# Autodesk Inventor assembly: BaseRoulante
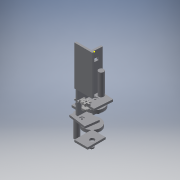
[picture p0: Inventor's stored thumbnail of the model, 180x180]
Saved by Autodesk Inventor 2017 SP1 (Build 210196100, 196)
## iProperties
Part Number: BaseRoulante
Material: Générique
Document SubType Name: Assembly
Designer: Sylvain
Author: Sylvain
## Documents named in this file (11)
- E:\1-SAUVEGARDE\Documents\Loisirs\GrosRobotOfficiel\3D\BaseRoulante.iam
- E:\1-SAUVEGARDE\Documents\Loisirs\GrosRobotOfficiel\3D\Flancs.ipt
- E:\1-SAUVEGARDE\Documents\Loisirs\GrosRobotOfficiel\3D\MoteurMaxon.ipt
- E:\1-SAUVEGARDE\Documents\Loisirs\GrosRobotOfficiel\3D\FlancExt.ipt
- E:\1-SAUVEGARDE\Documents\Loisirs\GrosRobotOfficiel\3D\Roue.ipt
- E:\1-SAUVEGARDE\Documents\Loisirs\GrosRobotOfficiel\3D\Base.ipt
- E:\1-SAUVEGARDE\Documents\Loisirs\GrosRobotOfficiel\3D\Roulement.ipt
- E:\1-SAUVEGARDE\Documents\Loisirs\GrosRobotOfficiel\3D\BaseRoulante\Design Accelerator\Engrenages cylindriques2.iam
- E:\1-SAUVEGARDE\Documents\Loisirs\GrosRobotOfficiel\3D\Toit.ipt
- E:\1-SAUVEGARDE\Documents\Loisirs\GrosRobotOfficiel\3D\BaseRoulante\Design Accelerator\Engrenages cylindriques4.iam
- E:\1-SAUVEGARDE\Documents\Loisirs\GrosRobotOfficiel\3D\BaseRoulante\Design Accelerator\Engrenages cylindriques5.iam
## Components (17 placed, 8 different names)
1. Flancs:1
2. Flancs:2 — Logement:1, Affleurement:1, Placage:1, Placage:2, Logement:3, Affleurement:2, Placage:4
3. MoteurMaxon:1 — Logement:3, Placage:3
4. MoteurMaxon:2
5. FlancExt:1
6. FlancExt:2 — Logement:2
7. Roue:1
8. Roue:2 — Cylindrique:1, Affleurement:2, Placage:5, Placage:6
9. Base:1 — Affleurement:1, Placage:1, Placage:2
10. Roulement:1 — Logement:1, Cylindrique:1
11. Roulement:2 — Logement:2
12. Roulement:3
13. Roulement:4
14. Engrenages cylindriques:1 [sub-assembly]
15. Toit:1
16. Engrenages cylindriques:2 [sub-assembly] — Placage:3, Placage:4, Placage:5, Placage:6
17. Engrenages cylindriques:3 [sub-assembly]
## Relationships (12: Mate 6, Insert 3, Flush 2, CylindricalJoint 1)
- Logement:1 [Insert]: Flancs:2 ↔ Roulement:1
- Logement:2 [Insert]: FlancExt:2 ↔ Roulement:2
- Affleurement:1 [Flush]: Flancs:2 ↔ Base:1
- Placage:1 [Mate]: Flancs:2 ↔ Base:1
- Placage:2 [Mate]: Flancs:2 ↔ Base:1
- Logement:3 [Insert]: Flancs:2 ↔ MoteurMaxon:1
- Cylindrique:1: Roue:2 ↔ Roulement:1
- Affleurement:2 [Flush]: Flancs:2 ↔ Roue:2
- Placage:3 [Mate]: MoteurMaxon:1 ↔ Engrenages cylindriques:2
- Placage:4 [Mate]: Flancs:2 ↔ Engrenages cylindriques:2
- Placage:5 [Mate]: Roue:2 ↔ Engrenages cylindriques:2
- Placage:6 [Mate]: Roue:2 ↔ Engrenages cylindriques:2
